# Autodesk Inventor assembly: Сборка1
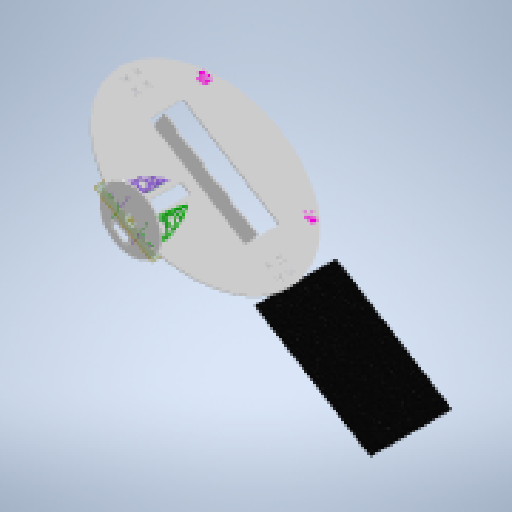
[picture p0: Inventor's stored thumbnail of the model, 512x512]
Saved by Autodesk Inventor 2023 (Build 270158000, 158)
## iProperties
Created: 2025-02-03
Part Number: Сборка1
Document SubType Name: Assembly
Designer: baranovaem
Author: baranovaem
## Documents named in this file (10)
- D:\лицо\Сборка1.iam
- D:\лицо\лицо1.ipt
- D:\лицо\магнит_стойка.ipt
- D:\лицо\монитор.ipt
- C:\Users\baranovaem\Downloads\экс\стенка.ipt
- D:\лицо\основа_лица.ipt
- D:\лицо\парус1.ipt
- D:\лицо\стенкаB.ipt
- D:\лицо\парус2.ipt
- \\sch239.net\UserHomes\Students\other\baranovaem\cheburashka\Cheburashka-main\Cheburashka_construction\platform\4ad8d019baf454c6bbd45c2c6ffb6783.ipt
## Components (17 placed, 9 different names)
1. лицо1:1 — Совмещение:1, Совмещение:2, Угол:1, Совмещение:68, Совмещение:69, Совмещение:70, Совмещение:72, Совмещение:73, Совмещение:74, Совмещение:76, Совмещение:78, Совмещение:79, Совмещение:82, Совмещение:84, Совмещение:85, Совмещение:86
2. магнит_стойка:1
3. магнит_стойка:2
4. магнит_стойка:3
5. магнит_стойка:4
6. монитор:1
7. стенка:1
8. основа_лица:1 — Совмещение:71, Совмещение:72, Совмещение:75, Совмещение:77, Совмещение:80
9. парус1:2 — Совмещение:68
10. парус1:4 — Совмещение:69, Совмещение:70
11. стенкаB:1
12. парус2:1
13. парус2:2
14. 4ad8d019baf454c6bbd45c2c6ffb6783:1 — Совмещение:71, Совмещение:73, Совмещение:84
15. 4ad8d019baf454c6bbd45c2c6ffb6783:2 — Совмещение:74, Совмещение:75, Совмещение:76, Совмещение:85
16. 4ad8d019baf454c6bbd45c2c6ffb6783:3 — Совмещение:77, Совмещение:78, Совмещение:82
17. 4ad8d019baf454c6bbd45c2c6ffb6783:4 — Совмещение:79, Совмещение:80, Совмещение:86
## Relationships (20: Mate 19, Angle 1)
- Совмещение:1 [Mate]: лицо1:1
- Совмещение:2 [Mate]: лицо1:1
- Угол:1 [Angle] (0 deg): лицо1:1
- Совмещение:68 [Mate]: лицо1:1 ↔ парус1:2
- Совмещение:69 [Mate]: лицо1:1 ↔ парус1:4
- Совмещение:70 [Mate]: лицо1:1 ↔ парус1:4
- Совмещение:71 [Mate]: основа_лица:1 ↔ 4ad8d019baf454c6bbd45c2c6ffb6783:1
- Совмещение:72 [Mate]: лицо1:1 ↔ основа_лица:1
- Совмещение:73 [Mate]: лицо1:1 ↔ 4ad8d019baf454c6bbd45c2c6ffb6783:1
- Совмещение:74 [Mate]: лицо1:1 ↔ 4ad8d019baf454c6bbd45c2c6ffb6783:2
- Совмещение:75 [Mate]: основа_лица:1 ↔ 4ad8d019baf454c6bbd45c2c6ffb6783:2
- Совмещение:76 [Mate]: лицо1:1 ↔ 4ad8d019baf454c6bbd45c2c6ffb6783:2
- Совмещение:77 [Mate]: основа_лица:1 ↔ 4ad8d019baf454c6bbd45c2c6ffb6783:3
- Совмещение:78 [Mate]: лицо1:1 ↔ 4ad8d019baf454c6bbd45c2c6ffb6783:3
- Совмещение:79 [Mate]: лицо1:1 ↔ 4ad8d019baf454c6bbd45c2c6ffb6783:4
- Совмещение:80 [Mate]: основа_лица:1 ↔ 4ad8d019baf454c6bbd45c2c6ffb6783:4
- Совмещение:82 [Mate]: лицо1:1 ↔ 4ad8d019baf454c6bbd45c2c6ffb6783:3
- Совмещение:84 [Mate]: лицо1:1 ↔ 4ad8d019baf454c6bbd45c2c6ffb6783:1
- Совмещение:85 [Mate]: лицо1:1 ↔ 4ad8d019baf454c6bbd45c2c6ffb6783:2
- Совмещение:86 [Mate]: лицо1:1 ↔ 4ad8d019baf454c6bbd45c2c6ffb6783:4
